# Autodesk Inventor assembly: X_GANTRY
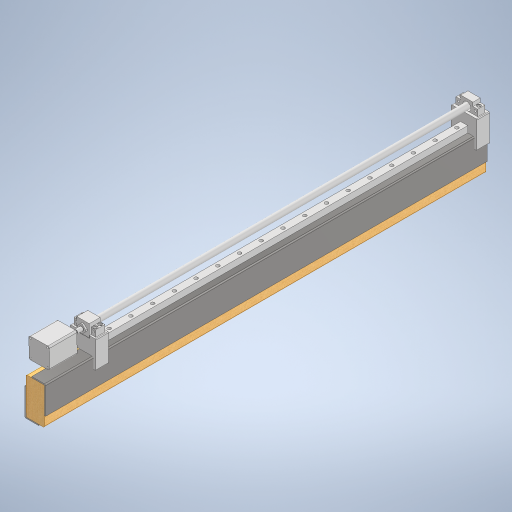
[picture p0: Inventor's stored thumbnail of the model, 512x512]
Saved by Autodesk Inventor 2023 (Build 270158000, 158)
## iProperties
Created: 2022-05-04
Part Number: X_GANTRY
Document SubType Name: Assembly
Designer: plebbb
Author: plebbb
## Documents named in this file (9)
- C:\Users\a laptop\Desktop\CNC_Project\X_GANTRY_WOOD.iam
- C:\Users\a laptop\Desktop\CNC_Project\HGW20CC_Rail_800mm.ipt
- C:\Users\a laptop\Desktop\CNC_Project\SFU1605_800mm.ipt
- C:\Users\a laptop\Desktop\CNC_Project\BF12.ipt
- C:\Users\a laptop\Desktop\CNC_Project\BK12.ipt
- C:\Users\a laptop\Desktop\CNC_Project\BK12_Spacer.ipt
- C:\Users\a laptop\Desktop\CNC_Project\BF12_Spacer.ipt
- C:\Users\a laptop\Desktop\CNC_Project\Nema23.ipt
- C:\Users\a laptop\Desktop\CNC_Project\Wood_X_Frame.iam
## Components (8 placed, 8 different names)
1. HGW20CC_Rail_800mm:1 — Mate:16, Flush:4
2. SFU1605_800mm:1
3. BF12:1
4. BK12:1
5. BK12_Spacer:1 — Mate:17, Mate:19
6. BF12_Spacer:1 — Flush:3, Mate:18
7. Nema23:1
8. Wood_X_Frame:1 [sub-assembly] — Flush:3, Mate:16, Mate:17, Mate:18, Mate:19, Flush:4
## Relationships (18: Mate 15, Flush 3)
- [Mate]: SFU1605_800mm:1 ↔ BK12:1
- [Flush]: SFU1605_800mm:1 ↔ BK12:1
- [Mate]: SFU1605_800mm:1 ↔ BF12:1
- [Mate]: SFU1605_800mm:1 ↔ BF12:1
- [Mate]: BK12:1 ↔ BK12_Spacer:1
- [Mate]: BK12:1 ↔ BK12_Spacer:1
- [Mate]: BK12:1 ↔ BK12_Spacer:1
- [Mate]: BF12:1 ↔ BF12_Spacer:1
- [Mate]: BF12:1 ↔ BF12_Spacer:1
- [Mate]: HGW20CC_Rail_800mm:1 ↔ BF12_Spacer:1
- [Mate]: SFU1605_800mm:1 ↔ Nema23:1
- [Mate]: SFU1605_800mm:1 ↔ Nema23:1
- Flush:3: BF12_Spacer:1 ↔ Wood_X_Frame:1
- Mate:16: HGW20CC_Rail_800mm:1 ↔ Wood_X_Frame:1
- Mate:17: BK12_Spacer:1 ↔ Wood_X_Frame:1
- Mate:18: BF12_Spacer:1 ↔ Wood_X_Frame:1
- Mate:19: BK12_Spacer:1 ↔ Wood_X_Frame:1
- Flush:4 (15.4 mm): HGW20CC_Rail_800mm:1 ↔ Wood_X_Frame:1
